# Autodesk Inventor assembly: sensor_chumacera
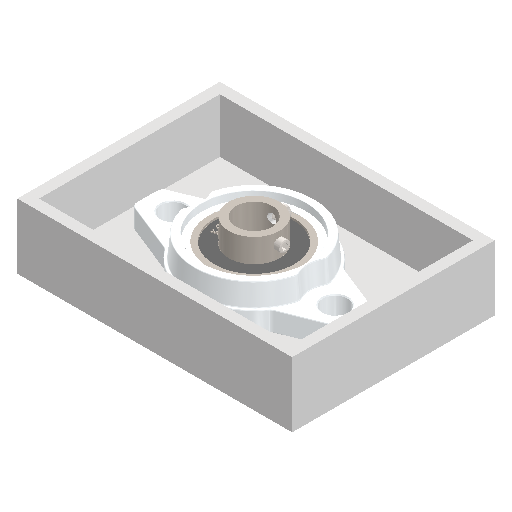
[picture p0: Inventor's stored thumbnail of the model, 512x512]
Saved by Autodesk Inventor 2025 (Build 290162000, 162)
## iProperties
Created: 2026-02-02
Part Number: sensor_chumacera
Document SubType Name: Assembly
Designer: HP
Author: HP
## Documents named in this file (3)
- C:\Users\HP\Desktop\CAD\sensor_chumacera.iam
- C:\Users\HP\Desktop\CAD\KFL000 bearing unit 10mm\KFL000 bearing unit 10mm.iam
- C:\Users\HP\Desktop\CAD\TORNILLO ALLEN CABEZA PLANA M3x0.5x6\estructura_sensor_chumacera.ipt
## Components (2 placed, 2 different names)
1. KFL000 bearing unit 10mm:1 [sub-assembly] — Nivelación:1
2. estructura_sensor_chumacera:1 — Nivelación:1
## Relationships (1: Flush 1)
- Nivelación:1 [Flush]: KFL000 bearing unit 10mm:1 ↔ estructura_sensor_chumacera:1
